# Autodesk Inventor assembly: Connettore adattatore e strip
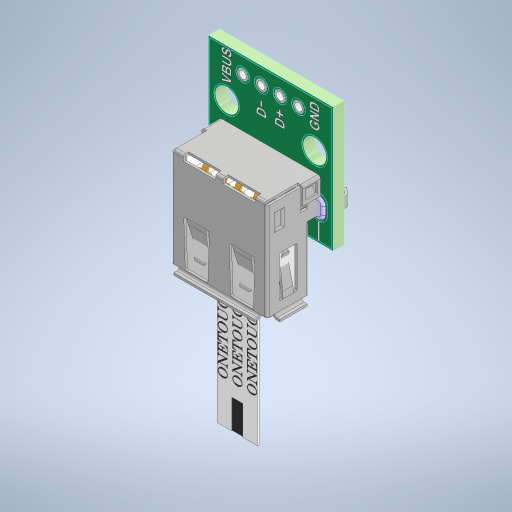
[picture p0: Inventor's stored thumbnail of the model, 512x512]
Saved by Autodesk Inventor 2023 (Build 270158000, 158)
## iProperties
Created: 2023-02-12
Part Number: Connettore adattatore e strip
Document SubType Name: Assembly
Designer: Gabriele
Author: Gabriele
## Documents named in this file (4)
- C:\Users\Gabriele\Desktop\LAB\AY2223_I_Project-2\3D\Case - Inventor\Connettore adattatore e strip.iam
- C:\Users\Gabriele\Desktop\LAB\AY2223_I_Project-2\3D\Case - Inventor\USB2A_Female_DIP2,54_PCB_adapter board.ipt
- C:\Users\Gabriele\Desktop\LAB\AY2223_I_Project-2\3D\Case - Inventor\Adattatore.ipt
- C:\Users\Gabriele\Desktop\LAB\AY2223_I_Project-2\3D\Case - Inventor\Strip.ipt
## Components (3 placed, 3 different names)
1. USB2A_Female_DIP2,54_PCB_adapter board:1 — Allineato:1, Coincidente:1, Coincidente:2, Coincidente:3
2. Adattatore:1 — Allineato:1, Coincidente:1, Coincidente:2, Coincidente:4, Coincidente:5
3. Strip:1 — Coincidente:3, Coincidente:4, Coincidente:5
## Relationships (6: Mate 5, Flush 1)
- Allineato:1 [Flush] (-9 mm): USB2A_Female_DIP2,54_PCB_adapter board:1 ↔ Adattatore:1
- Coincidente:1 [Mate] (0.2 mm): USB2A_Female_DIP2,54_PCB_adapter board:1 ↔ Adattatore:1
- Coincidente:2 [Mate] (0.2 mm): USB2A_Female_DIP2,54_PCB_adapter board:1 ↔ Adattatore:1
- Coincidente:3 [Mate] (0.2 mm): USB2A_Female_DIP2,54_PCB_adapter board:1 ↔ Strip:1
- Coincidente:4 [Mate] (0.1 mm): Adattatore:1 ↔ Strip:1
- Coincidente:5 [Mate] (0.2 mm): Adattatore:1 ↔ Strip:1
